# Autodesk Inventor assembly: beam_sub_asssem
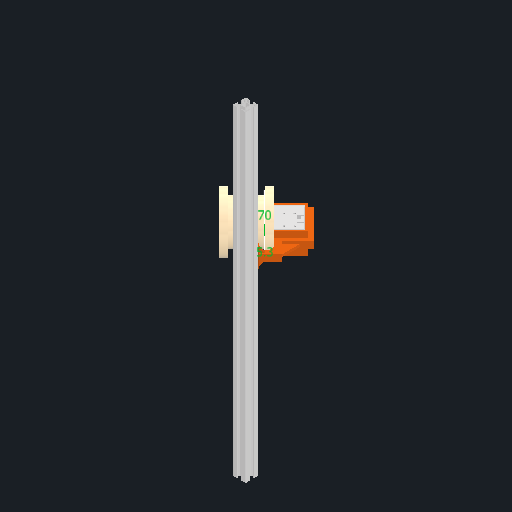
[picture p0: Inventor's stored thumbnail of the model, 512x512]
Saved by Autodesk Inventor 2026.2 (Build 302298010, 298A)
## iProperties
Created: 2026-02-11
Part Number: beam_sub_asssem
Document SubType Name: Assembly
Designer: Luke
Mass: 458.356 g
Surface Area: 1751.66 cm^2
Volume: 311.662 cm^3
Density: 1.47068 g/cm^3
Author: Luke
## Documents named in this file (6)
- C:\Users\Luke\OneDrive - Heriot-Watt University\Desktop\Robot Mech Sys\GroupProject\CAD\sub_assemblies\beam_sub_asssem.iam
- C:\Users\Luke\OneDrive - Heriot-Watt University\Desktop\Robot Mech Sys\GroupProject\CAD\parts\SIDE_BEAMS.ipt
- C:\Users\Luke\OneDrive - Heriot-Watt University\Desktop\Robot Mech Sys\GroupProject\CAD\sub_assemblies\motor_mount_sub_assem.iam
- C:\Users\Luke\Documents\Inventor\Content Center Files\R2026\en-US\BS EN ISO 7045 H\EN ISO 7045 - M2 x 10 - 4.8 - H(1).ipt
- C:\Users\Luke\Documents\Inventor\Content Center Files\R2026\en-US\BS EN 24032\ISO 4032 - M2BS EN.ipt
- C:\Users\Luke\Documents\Inventor\Content Center Files\R2026\en-US\BS EN 24032\ISO 4032 - M2.5BS EN.ipt
## Components (6 placed, 5 different names)
1. SIDE_BEAMS:1 — Mate:1, Mate:2, Mate:3
2. motor_mount_sub_assem:1 [sub-assembly] — Mate:1, Mate:2, Mate:3, Insert:1, Mate:6, Mate:8
3. BS EN ISO 7045 H - Metric M2 x 10 - 4.8 - H:1
4. BS EN ISO 7045 H - Metric M2 x 10 - 4.8 - H:2 — Mate:6, Mate:7, Mate:8
5. BS EN 24032 - Metric M2.5:1 — Insert:1
6. BS EN 24032 - Metric M2:1 — Mate:7
## Relationships (8: Mate 7, Insert 1)
- Mate:1 (0.2 mm): SIDE_BEAMS:1 ↔ motor_mount_sub_assem:1
- Mate:2 (0.2 mm): SIDE_BEAMS:1 ↔ motor_mount_sub_assem:1
- Mate:3 (0.6 mm): SIDE_BEAMS:1 ↔ motor_mount_sub_assem:1
- [Mate]: motor_mount_sub_assem:1 ↔ BS EN ISO 7045 H - Metric M2 x 10 - 4.8 - H:1
- Insert:1: motor_mount_sub_assem:1 ↔ BS EN 24032 - Metric M2.5:1
- Mate:6: motor_mount_sub_assem:1 ↔ BS EN ISO 7045 H - Metric M2 x 10 - 4.8 - H:2
- Mate:7: BS EN ISO 7045 H - Metric M2 x 10 - 4.8 - H:2 ↔ BS EN 24032 - Metric M2:1
- Mate:8: motor_mount_sub_assem:1 ↔ BS EN ISO 7045 H - Metric M2 x 10 - 4.8 - H:2
